# Autodesk Inventor assembly: frame
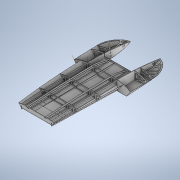
[picture p0: Inventor's stored thumbnail of the model, 180x180]
Saved by Autodesk Inventor 2022 (Build 260153000, 153)
## iProperties
Created: 2021-04-24
Part Number: frame
Document SubType Name: Assembly
Designer: kardo
Mass: 203.812 g
Surface Area: 2196.1 cm^2
Volume: 203.812 cm^3
Density: 1 g/cm^3
Author: kardo
## Documents named in this file (23)
- D:\Computer Aided Design\hydroplane_plan_2\assembly\frame.iam
- D:\Computer Aided Design\hydroplane_plan_2\frame_parts\stringer.ipt
- D:\Computer Aided Design\hydroplane_plan_2\frame_parts\bulkhead_main.ipt
- D:\Computer Aided Design\hydroplane_plan_2\frame_parts\bulkhead_transom.ipt
- D:\Computer Aided Design\hydroplane_plan_2\frame_parts\bulkhead_b1.ipt
- D:\Computer Aided Design\hydroplane_plan_2\frame_parts\bulkhead_b2.ipt
- D:\Computer Aided Design\hydroplane_plan_2\frame_parts\bulkhead_front_center.ipt
- D:\Computer Aided Design\hydroplane_plan_2\frame_parts\aux_nose_side.ipt
- D:\Computer Aided Design\hydroplane_plan_2\frame_parts\bulkhead_sponson_break.ipt
- D:\Computer Aided Design\hydroplane_plan_2\frame_parts\aux_nose_bottom.ipt
- D:\Computer Aided Design\hydroplane_plan_2\frame_parts\aux_nose_bottom_bracket.ipt
- D:\Computer Aided Design\hydroplane_plan_2\frame_parts\aux_nose_side_bracket.ipt
- D:\Computer Aided Design\hydroplane_plan_2\frame_parts\standoff.ipt
- D:\Computer Aided Design\hydroplane_plan_2\frame_parts\cowl_liner.ipt
- D:\Computer Aided Design\hydroplane_plan_2\frame_parts\stringer_cowl.ipt
- D:\Computer Aided Design\hydroplane_plan_2\shell_parts\deck.ipt
- D:\Computer Aided Design\hydroplane_plan_2\shell_parts\tunnel_side.ipt
- D:\Computer Aided Design\hydroplane_plan_2\shell_parts\tunnel_center.ipt
- D:\Computer Aided Design\hydroplane_plan_2\shell_parts\tail_side.ipt
- D:\Computer Aided Design\hydroplane_plan_2\shell_parts\sponson_bottom.ipt
- D:\Computer Aided Design\hydroplane_plan_2\shell_parts\sponson_side.ipt
- D:\Computer Aided Design\hydroplane_plan_2\assembly\sponson_bottom_MIR1.ipt
- D:\Computer Aided Design\hydroplane_plan_2\assembly\sponson_side_MIR1.ipt
## Components (35 placed, 22 different names)
1. stringer:1 — Mate:4, Mate:5, Mate:6, Mate:62, Mate:63, Mate:64, Mate:65, Mate:66, Mate:67, Mate:96
2. stringer:2 — Mate:1, Mate:2, Mate:3, Mate:7, Mate:8, Mate:9, Mate:10, Mate:11, Mate:12, Mate:13, Mate:14, Mate:15, Mate:16, Mate:17, Mate:18, Mate:19, Mate:20, Mate:21, Mate:34, Mate:35, Mate:36, Mate:37, Mate:88
3. bulkhead_main:1 — Mate:1, Mate:2, Mate:3, Mate:4, Mate:5, Mate:6, Mate:42, Mate:43, Mate:50, Mate:51, Mate:52, Mate:53, Mate:60, Mate:61, Mate:76, Mate:77, Mate:90, Mate:91, Mate:92, Mate:93, Mate:97, Mate:98, Mate:99, Mate:100
4. bulkhead_transom:1 — Mate:7, Mate:8, Mate:9, Mate:45, Mate:49, Mate:58, Mate:59, Mate:80, Mate:83, Mate:84, Mate:86, Mate:94
5. bulkhead_b1:1 — Mate:11, Mate:13, Mate:15, Mate:87, Mate:95
6. bulkhead_b2:1 — Mate:10, Mate:12, Mate:14
7. bulkhead_front_center:1 — Mate:16, Mate:17, Mate:18, Mate:44, Mate:46, Mate:47, Mate:48, Mate:54, Mate:55, Mate:56, Mate:57, Mate:78, Mate:79, Mate:81, Mate:82, Mate:85
8. aux_nose_side:1 — Mate:30, Mate:31, Mate:40
9. bulkhead_sponson_break:1 — Mate:19, Mate:20, Mate:21, Mate:25, Mate:27, Mate:30, Mate:31
10. aux_nose_bottom:1 — Mate:25, Mate:27, Mate:41
11. aux_nose_bottom_bracket:1 — Mate:34, Mate:36, Mate:39
12. aux_nose_side_bracket:1 — Mate:35, Mate:37, Mate:38
13. standoff:1 — Mate:42, Mate:43, Flush:1
14. cowl_liner:1 — Mate:44, Mate:45, Mate:46
15. cowl_liner:2 — Mate:47, Mate:48, Mate:49
16. stringer_cowl:1 — Mate:50, Mate:51
17. standoff:2 — Mate:52, Mate:53
18. cowl_liner:3 — Mate:55, Mate:57, Mate:59
19. cowl_liner:4 — Mate:54, Mate:56, Mate:58
20. stringer_cowl:2 — Mate:60, Mate:61
21. bulkhead_sponson_break:2 — Mate:62, Mate:63, Mate:68, Mate:69, Mate:73, Mate:74
22. aux_nose_side:2 — Mate:68, Mate:69, Mate:72
23. aux_nose_bottom:2 — Mate:73, Mate:74, Mate:75
24. aux_nose_side_bracket:2 — Mate:64, Mate:65, Mate:70
25. aux_nose_bottom_bracket:2 — Mate:66, Mate:67, Mate:71
26. deck:1 — Mate:76, Mate:77
27. tunnel_side:1 — Mate:78, Mate:79, Mate:80
28. tunnel_side:2 — Mate:81, Mate:82, Mate:83
29. tunnel_center:1 — Mate:84, Mate:85, Flush:1
30. tail_side:1 — Mate:86, Mate:87, Mate:88
31. sponson_bottom:1 — Mate:90, Mate:91
32. sponson_side:1 — Mate:92, Mate:93
33. tail_side:2 — Mate:94, Mate:95, Mate:96
34. sponson_bottom_MIR:1 — Mate:97, Mate:98
35. sponson_side_MIR:1 — Mate:99, Mate:100
## Relationships (92: Mate 91, Flush 1)
- Mate:1: stringer:2 ↔ bulkhead_main:1
- Mate:2: stringer:2 ↔ bulkhead_main:1
- Mate:3: stringer:2 ↔ bulkhead_main:1
- Mate:4: stringer:1 ↔ bulkhead_main:1
- Mate:5: stringer:1 ↔ bulkhead_main:1
- Mate:6: stringer:1 ↔ bulkhead_main:1
- Mate:7: stringer:2 ↔ bulkhead_transom:1
- Mate:8: stringer:2 ↔ bulkhead_transom:1
- Mate:9: stringer:2 ↔ bulkhead_transom:1
- Mate:10: stringer:2 ↔ bulkhead_b2:1
- Mate:11: stringer:2 ↔ bulkhead_b1:1
- Mate:12: stringer:2 ↔ bulkhead_b2:1
- Mate:13: stringer:2 ↔ bulkhead_b1:1
- Mate:14: stringer:2 ↔ bulkhead_b2:1
- Mate:15: stringer:2 ↔ bulkhead_b1:1
- Mate:16: stringer:2 ↔ bulkhead_front_center:1
- Mate:17: stringer:2 ↔ bulkhead_front_center:1
- Mate:18: stringer:2 ↔ bulkhead_front_center:1
- Mate:19: stringer:2 ↔ bulkhead_sponson_break:1
- Mate:20: stringer:2 ↔ bulkhead_sponson_break:1
- Mate:21: stringer:2 ↔ bulkhead_sponson_break:1
- Mate:25: bulkhead_sponson_break:1 ↔ aux_nose_bottom:1
- Mate:27: bulkhead_sponson_break:1 ↔ aux_nose_bottom:1
- Mate:30: aux_nose_side:1 ↔ bulkhead_sponson_break:1
- Mate:31: aux_nose_side:1 ↔ bulkhead_sponson_break:1
- Mate:34: stringer:2 ↔ aux_nose_bottom_bracket:1
- Mate:35: stringer:2 ↔ aux_nose_side_bracket:1
- Mate:36: stringer:2 ↔ aux_nose_bottom_bracket:1
- Mate:37: stringer:2 ↔ aux_nose_side_bracket:1
- Mate:38: aux_nose_side_bracket:1
- Mate:39: aux_nose_bottom_bracket:1
- Mate:40: aux_nose_side:1
- Mate:41: aux_nose_bottom:1
- Mate:42: bulkhead_main:1 ↔ standoff:1
- Mate:43: bulkhead_main:1 ↔ standoff:1
- Mate:44: bulkhead_front_center:1 ↔ cowl_liner:1
- Mate:45: bulkhead_transom:1 ↔ cowl_liner:1
- Mate:46: bulkhead_front_center:1 ↔ cowl_liner:1
- Mate:47: bulkhead_front_center:1 ↔ cowl_liner:2
- Mate:48: bulkhead_front_center:1 ↔ cowl_liner:2
- Mate:49: bulkhead_transom:1 ↔ cowl_liner:2
- Mate:50: bulkhead_main:1 ↔ stringer_cowl:1
- Mate:51: bulkhead_main:1 ↔ stringer_cowl:1
- Mate:52: bulkhead_main:1 ↔ standoff:2
- Mate:53: bulkhead_main:1 ↔ standoff:2
- Mate:54: bulkhead_front_center:1 ↔ cowl_liner:4
- Mate:55: bulkhead_front_center:1 ↔ cowl_liner:3
- Mate:56: bulkhead_front_center:1 ↔ cowl_liner:4
- Mate:57: bulkhead_front_center:1 ↔ cowl_liner:3
- Mate:58: bulkhead_transom:1 ↔ cowl_liner:4
- Mate:59: bulkhead_transom:1 ↔ cowl_liner:3
- Mate:60: bulkhead_main:1 ↔ stringer_cowl:2
- Mate:61: bulkhead_main:1 ↔ stringer_cowl:2
- Mate:62: stringer:1 ↔ bulkhead_sponson_break:2
- Mate:63: stringer:1 ↔ bulkhead_sponson_break:2
- Mate:64: stringer:1 ↔ aux_nose_side_bracket:2
- Mate:65: stringer:1 ↔ aux_nose_side_bracket:2
- Mate:66: stringer:1 ↔ aux_nose_bottom_bracket:2
- Mate:67: stringer:1 ↔ aux_nose_bottom_bracket:2
- Mate:68: bulkhead_sponson_break:2 ↔ aux_nose_side:2
- Mate:69: bulkhead_sponson_break:2 ↔ aux_nose_side:2
- Mate:70: aux_nose_side_bracket:2
- Mate:71: aux_nose_bottom_bracket:2
- Mate:72: aux_nose_side:2
- Mate:73: bulkhead_sponson_break:2 ↔ aux_nose_bottom:2
- Mate:74: bulkhead_sponson_break:2 ↔ aux_nose_bottom:2
- Mate:75: aux_nose_bottom:2
- Mate:76: bulkhead_main:1 ↔ deck:1
- Mate:77: bulkhead_main:1 ↔ deck:1
- Mate:78: bulkhead_front_center:1 ↔ tunnel_side:1
- Mate:79: bulkhead_front_center:1 ↔ tunnel_side:1
- Mate:80: bulkhead_transom:1 ↔ tunnel_side:1
- Mate:81: bulkhead_front_center:1 ↔ tunnel_side:2
- Mate:82: bulkhead_front_center:1 ↔ tunnel_side:2
- Mate:83: bulkhead_transom:1 ↔ tunnel_side:2
- Mate:84: bulkhead_transom:1 ↔ tunnel_center:1
- Mate:85: bulkhead_front_center:1 ↔ tunnel_center:1
- Flush:1: standoff:1 ↔ tunnel_center:1
- Mate:86: bulkhead_transom:1 ↔ tail_side:1
- Mate:87: bulkhead_b1:1 ↔ tail_side:1
- Mate:88: stringer:2 ↔ tail_side:1
- Mate:90: bulkhead_main:1 ↔ sponson_bottom:1
- Mate:91: bulkhead_main:1 ↔ sponson_bottom:1
- Mate:92: bulkhead_main:1 ↔ sponson_side:1
- Mate:93: bulkhead_main:1 ↔ sponson_side:1
- Mate:94: bulkhead_transom:1 ↔ tail_side:2
- Mate:95: bulkhead_b1:1 ↔ tail_side:2
- Mate:96: stringer:1 ↔ tail_side:2
- Mate:97: bulkhead_main:1 ↔ sponson_bottom_MIR:1
- Mate:98: bulkhead_main:1 ↔ sponson_bottom_MIR:1
- Mate:99: bulkhead_main:1 ↔ sponson_side_MIR:1
- Mate:100: bulkhead_main:1 ↔ sponson_side_MIR:1
